# Autodesk Inventor assembly: airhockeybot_y_simulation_centered
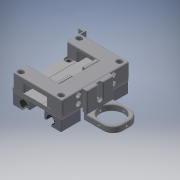
[picture p0: Inventor's stored thumbnail of the model, 180x180]
Saved by Autodesk Inventor 2019.3 (Build 233278000, 278)
## iProperties
Created: 2020-12-03
Part Number: airhockeybot_y_simulation_centered
Material: Generisch
Document SubType Name: Assembly
Designer: Nicolas Frick
Mass: 155.059 g
Surface Area: 651.892 cm^2
Volume: 155.059 cm^3
Density: 1 g/cm^3
Author: Nicolas Frick
## Documents named in this file (2)
- C:\Users\Nicolas Frick\Sync\OneDrive\airhockeybot\mechanical_design\common_cad_parts\sim_models\airhockeybot_y_simulation_centered.iam
- C:\Users\Nicolas Frick\Sync\OneDrive\airhockeybot\mechanical_design\common_cad_parts\sim_models\airhockeybot_y_simulation.iam
## Components (1 placed, 1 different names)
1. airhockeybot_y_simulation:1 [sub-assembly] — Passend:1, Fluchtend:1, Passend:2
## Relationships (3: Mate 2, Flush 1)
- Passend:1 [Mate] (-10 mm): airhockeybot_y_simulation:1
- Fluchtend:1 [Flush] (-64 mm): airhockeybot_y_simulation:1
- Passend:2 [Mate] (-36 mm): airhockeybot_y_simulation:1
